# Autodesk Inventor assembly: ASY MSC 002 отстойник осветлитель
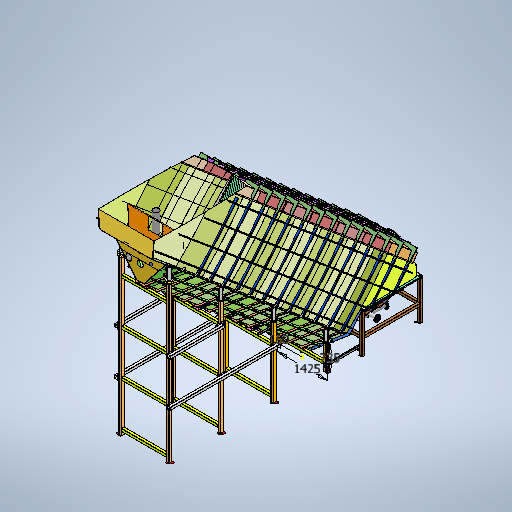
[picture p0: Inventor's stored thumbnail of the model, 512x512]
Saved by Autodesk Inventor 2025 (Build 290162010, 162A)
## iProperties
Created: 2024-09-05
Part Number: ASY MSC 002 отстойник осветлитель
Document SubType Name: Assembly
Designer: admin
Author: admin
## Documents named in this file (33)
- C:\Users\admin\YandexDisk-badmisterfox\домашниий пк\Inventor\Manturovo\Manturovo_Se-clar\ASY MSC 002 отстойник осветлитель.iam
- C:\Users\admin\YandexDisk-badmisterfox\домашниий пк\Inventor\Manturovo\Manturovo_Se-clar\ASY MSC 900.1 base frame.iam
- C:\Users\admin\YandexDisk-badmisterfox\домашниий пк\Inventor\Manturovo\Manturovo_Se-clar\ASY MSC 100 cone.iam
- C:\Users\admin\YandexDisk-badmisterfox\домашниий пк\Inventor\Manturovo\Manturovo_Se-clar\MSC 401 sheet lowerback.ipt
- C:\Users\admin\YandexDisk-badmisterfox\домашниий пк\Inventor\Manturovo\Manturovo_Se-clar\MSC 701 face 1.ipt
- C:\Users\admin\YandexDisk-badmisterfox\домашниий пк\Inventor\Manturovo\Manturovo_Se-clar\MSC 705 ridge 3.ipt
- C:\Users\admin\YandexDisk-badmisterfox\домашниий пк\Inventor\Manturovo\Manturovo_Se-clar\MSC 713 tube.ipt
- C:\Users\admin\YandexDisk-badmisterfox\домашниий пк\Inventor\Manturovo\Manturovo_Se-clar\ISO 5251 Bends 3D without straight ends(90 deg) DN150 11 11.ipt
- C:\Users\admin\YandexDisk-badmisterfox\домашниий пк\Inventor\Manturovo\Manturovo_Se-clar\MSC 408 stringer lowerback.ipt
- C:\Users\admin\YandexDisk-badmisterfox\домашниий пк\Inventor\Manturovo\Manturovo_Se-clar\MSC 703 face 2.ipt
- C:\Users\admin\YandexDisk-badmisterfox\домашниий пк\Inventor\Manturovo\Manturovo_Se-clar\MSC 702 face 3.ipt
- C:\Users\admin\YandexDisk-badmisterfox\домашниий пк\Inventor\Manturovo\Manturovo_Se-clar\MSC 704 face 4.ipt
- C:\Users\admin\YandexDisk-badmisterfox\домашниий пк\Inventor\Manturovo\Manturovo_Se-clar\ASY MSC 900.3 base frame.iam
- C:\Users\admin\YandexDisk-badmisterfox\домашниий пк\Inventor\Manturovo\Manturovo_Se-clar\Pillars\ASY MSC 900.5 base frame.iam
- C:\Users\admin\YandexDisk-badmisterfox\домашниий пк\Inventor\Manturovo\Manturovo_Se-clar\Pillars\ASY MSC 900.4  base frame.iam
- C:\Users\admin\YandexDisk-badmisterfox\домашниий пк\Inventor\Manturovo\Manturovo_Se-clar\Pillars\ASY MSC 900.6 base frame.iam
- C:\Users\admin\YandexDisk-badmisterfox\домашниий пк\Inventor\Manturovo\Manturovo_Se-clar\ASY MSC 200 BACK.iam
- C:\Users\admin\YandexDisk-badmisterfox\домашниий пк\Inventor\Manturovo\Manturovo_Se-clar\ASY MSC 300.2 LEFT BOARD.iam
- C:\Users\admin\YandexDisk-badmisterfox\домашниий пк\Inventor\Manturovo\Manturovo_Se-clar\ASY MSC 300.1 RIGHT BOARD.iam
- C:\Users\admin\YandexDisk-badmisterfox\домашниий пк\Inventor\Manturovo\Manturovo_Se-clar\ASY MSC 500 BELLY.iam
- C:\Users\admin\YandexDisk-badmisterfox\домашниий пк\Inventor\Manturovo\Manturovo_Se-clar\ASY MSC 900.2 support.iam
- C:\Users\admin\YandexDisk-badmisterfox\домашниий пк\Inventor\Manturovo\Manturovo_Se-clar\ASY MSC 600 cone exit back.iam
- C:\Users\admin\YandexDisk-badmisterfox\домашниий пк\Inventor\Manturovo\Manturovo_Se-clar\ASY MSC 800 gills.iam
- C:\Users\admin\YandexDisk-badmisterfox\домашниий пк\Inventor\Manturovo\Manturovo_Se-clar\ASY MSC 400 Accsess hatch.iam
- C:\Users\admin\YandexDisk-badmisterfox\домашниий пк\Inventor\Manturovo\Manturovo_Se-clar\MSC DIM 000 settler-clarifier.ipt
- C:\Users\admin\YandexDisk-badmisterfox\домашниий пк\Inventor\Manturovo\Manturovo_Se-clar\MSC DIM 001 frame.ipt
- C:\Users\admin\YandexDisk-badmisterfox\домашниий пк\Inventor\Manturovo\Manturovo_Se-clar\ASY MSC 900.7 base frame transverse.iam
- C:\Users\admin\YandexDisk-badmisterfox\домашниий пк\Inventor\Manturovo\Manturovo_Se-clar\ASY MSC 900.8 base frame transverse.iam
- C:\Users\admin\YandexDisk-badmisterfox\домашниий пк\Inventor\Manturovo\Manturovo_Se-clar\MSC 908 transverse pillar plate.ipt
- C:\Users\admin\YandexDisk-badmisterfox\домашниий пк\Inventor\Manturovo\Manturovo_Se-clar\Part2.ipt
- C:\Users\admin\YandexDisk-badmisterfox\домашниий пк\Inventor\Manturovo\Manturovo_Se-clar\MSC 900.9 base frame transverse.ipt
- C:\Users\admin\YandexDisk-badmisterfox\домашниий пк\Inventor\Manturovo\Manturovo_Se-clar\ASY MSC 700 water tray.iam
- C:\Users\admin\YandexDisk-badmisterfox\домашниий пк\Inventor\Manturovo\Manturovo_Se-clar\ASY 940 linkage.iam
## Components (51 placed, 32 different names)
1. MSC DIM 000 settler-clarifier:1
2. MSC DIM 001 frame:1
3. ASY MSC 900.1 base frame:1 [sub-assembly] — Flush:4, Mate:18, Flush:5, Mate:19, Mate:44, Mate:47, Mate:50, Flush:16
4. ASY MSC 100 cone:1 [sub-assembly] — Mate:19, Flush:6, Mate:29, Rigid:17
5. MSC 401 sheet lowerback:1 — Mate:29, Mate:30, Mate:31
6. MSC 701 face 1:1 — Rigid:4, Flush:9, Mate:35
7. MSC 705 ridge 3:1
8. MSC 713 tube:1 — Rigid:4
9. ISO 5251 Bends 3D without straight ends(90 deg) DN150 11:1
10. MSC 408 stringer lowerback:1
11. MSC 713 tube:2
12. MSC 703 face 2:1 — Flush:13, Flush:17, Mate:66
13. MSC 702 face 3:1 — Mate:34, Mate:35, Mate:36, Mate:66
14. MSC 704 face 4:1
15. MSC 408 stringer lowerback:2
16. ASY MSC 900.3 base frame:1 [sub-assembly] — Mate:23, Mate:24, Cylindrical:4, Mate:44, Mate:45, Rigid:26, Rigid:31, Rigid:32
17. ASY MSC 900.5 base frame:1 [sub-assembly] — Flush:11, Cylindrical:7, Cylindrical:8, Mate:46, Mate:48, Rigid:28
18. ASY MSC 900.4  base frame:1 [sub-assembly] — Mate:32, Mate:33, Mate:45, Mate:46, Rigid:27
19. ASY MSC 900.6 base frame:1 [sub-assembly] — Mate:38, Mate:39, Cylindrical:5, Cylindrical:6, Mate:47, Rigid:19, Rigid:20, Rigid:21, Rigid:22, Rigid:29
20. ASY MSC 200 BACK:1 [sub-assembly] — Flush:8, Mate:31
21. ASY MSC 300.2 LEFT BOARD:1 [sub-assembly] — Rigid:11, Mate:34
22. ASY MSC 300.1 RIGHT BOARD:1 [sub-assembly] — Rigid:10, Flush:17
23. ASY MSC 500 BELLY:1 [sub-assembly] — Flush:7, Mate:22, Mate:25, Rigid:10, Rigid:11, Mate:40, Mate:41, Mate:42, Mate:43
24. ASY MSC 900.2 support:1 [sub-assembly] — Cylindrical:8, Mate:40
25. ASY MSC 900.2 support:2 [sub-assembly]
26. ASY MSC 900.2 support:3 [sub-assembly] — Cylindrical:4, Mate:25
27. ASY MSC 900.2 support:4 [sub-assembly] — Cylindrical:6, Mate:42
28. ASY MSC 900.2 support:5 [sub-assembly]
29. ASY MSC 600 cone exit back:1 [sub-assembly] — Rigid:17
30. ASY MSC 800 gills:1 [sub-assembly] — Mate:22
31. ASY MSC 900.2 support:6 [sub-assembly] — Cylindrical:7, Mate:41
32. ASY MSC 900.2 support:7 [sub-assembly]
33. ASY MSC 400 Accsess hatch:1 [sub-assembly]
34. ASY MSC 900.2 support:8 [sub-assembly] — Cylindrical:5, Mate:43
35. ASY MSC 900.7 base frame transverse:1 [sub-assembly] — Rigid:19
36. ASY MSC 900.7 base frame transverse:2 [sub-assembly] — Rigid:20
37. ASY MSC 900.8 base frame transverse:1 [sub-assembly] — Rigid:21
38. ASY MSC 900.8 base frame transverse:2 [sub-assembly] — Rigid:22
39. MSC 908 transverse pillar plate:4 — Mate:50, Flush:16, Flush:18
40. Part2:1 — Rigid:26, Mate:51
41. MSC 900.9 base frame transverse:1 — Mate:51
42. Part2:2 — Rigid:27, Mate:59
43. MSC 900.9 base frame transverse:2 — Mate:59
44. Part2:3 — Rigid:28
45. MSC 900.9 base frame transverse:3
46. Part2:4 — Rigid:29
47. MSC 900.9 base frame transverse:4
48. ASY MSC 700 water tray:1 [sub-assembly]
49. ASY 940 linkage:1 [sub-assembly] — Rigid:32, Flush:18
50. MSC 908 transverse pillar plate:8
51. ASY 940 linkage:2 [sub-assembly] — Rigid:31
## Relationships (87: Mate 45, WeldJoint 19, Flush 14, CylindricalJoint 8, RevoluteJoint 1)
- [Mate]: ASY MSC 100 cone:1 ↔ MSC 401 sheet lowerback:1
- [WeldJoint]: MSC 713 tube:1 ↔ ISO 5251 Bends 3D without straight ends(90 deg) DN150 11:1
- [Mate]: ASY MSC 100 cone:1 ↔ MSC 408 stringer lowerback:1
- [RevoluteJoint]: ISO 5251 Bends 3D without straight ends(90 deg) DN150 11:1 ↔ MSC 713 tube:2
- Rigid:4 [WeldJoint]: MSC 701 face 1:1 ↔ MSC 713 tube:1
- [Mate]: ASY MSC 100 cone:1 ↔ MSC 408 stringer lowerback:2
- [Mate]: ASY MSC 500 BELLY:1 ↔ ASY MSC 600 cone exit back:1
- [Flush]: ASY MSC 900.1 base frame:1 ↔ ASY MSC 100 cone:1
- [WeldJoint]: MSC 705 ridge 3:1 ↔ ASY MSC 700 water tray:1
- [WeldJoint]: MSC 705 ridge 3:1 ↔ ASY MSC 700 water tray:1
- [Flush]: ASY MSC 500 BELLY:1 ↔ ASY MSC 600 cone exit back:1
- [Mate]: ASY MSC 500 BELLY:1 ↔ ASY MSC 800 gills:1
- [Mate]: MSC 701 face 1:1 ↔ ASY MSC 500 BELLY:1
- [Mate] (-5 mm): MSC 701 face 1:1 ↔ ASY MSC 500 BELLY:1
- [Mate] (3 mm): ASY MSC 500 BELLY:1 ↔ ASY MSC 900.2 support:2
- [Mate] (3 mm): ASY MSC 500 BELLY:1 ↔ ASY MSC 900.2 support:5
- [Mate] (3 mm): ASY MSC 500 BELLY:1 ↔ ASY MSC 900.2 support:7
- [CylindricalJoint]: ASY MSC 900.4  base frame:1 ↔ ASY MSC 900.2 support:5
- [CylindricalJoint]: ASY MSC 900.4  base frame:1 ↔ ASY MSC 900.2 support:2
- [Mate] (-2860 mm): ASY MSC 200 BACK:1 ↔ ASY MSC 500 BELLY:1
- [CylindricalJoint]: ASY MSC 900.3 base frame:1 ↔ ASY MSC 900.2 support:7
- [Flush]: ASY MSC 900.3 base frame:1 ↔ ASY MSC 900.4  base frame:1
- Flush:4: ASY MSC 900.1 base frame:1
- Mate:18 (4 mm): ASY MSC 900.1 base frame:1
- Flush:5: ASY MSC 900.1 base frame:1
- Mate:19: ASY MSC 900.1 base frame:1 ↔ ASY MSC 100 cone:1
- Flush:6: ASY MSC 100 cone:1
- Flush:7: ASY MSC 500 BELLY:1
- Flush:8: ASY MSC 200 BACK:1
- Mate:22: ASY MSC 500 BELLY:1 ↔ ASY MSC 800 gills:1
- Mate:23: ASY MSC 900.3 base frame:1
- Mate:24: ASY MSC 900.3 base frame:1
- Cylindrical:4: ASY MSC 900.3 base frame:1 ↔ ASY MSC 900.2 support:3
- Mate:25 (3 mm): ASY MSC 500 BELLY:1 ↔ ASY MSC 900.2 support:3
- Flush:9: MSC 701 face 1:1
- Mate:29: ASY MSC 100 cone:1 ↔ MSC 401 sheet lowerback:1
- Mate:30: MSC 401 sheet lowerback:1
- Mate:31: MSC 401 sheet lowerback:1 ↔ ASY MSC 200 BACK:1
- Rigid:10 [WeldJoint] (-25 mm): ASY MSC 300.1 RIGHT BOARD:1 ↔ ASY MSC 500 BELLY:1
- Rigid:11 [WeldJoint] (-25 mm): ASY MSC 300.2 LEFT BOARD:1 ↔ ASY MSC 500 BELLY:1
- Flush:11: ASY MSC 900.5 base frame:1
- Mate:32: ASY MSC 900.4  base frame:1
- Mate:33: ASY MSC 900.4  base frame:1
- Mate:34: MSC 702 face 3:1 ↔ ASY MSC 300.2 LEFT BOARD:1
- Mate:35: MSC 701 face 1:1 ↔ MSC 702 face 3:1
- [WeldJoint]: MSC 705 ridge 3:1 ↔ ASY MSC 700 water tray:1
- Mate:36: MSC 702 face 3:1
- Mate:38: ASY MSC 900.6 base frame:1
- Mate:39: ASY MSC 900.6 base frame:1
- Cylindrical:5: ASY MSC 900.6 base frame:1 ↔ ASY MSC 900.2 support:8
- Cylindrical:6: ASY MSC 900.6 base frame:1 ↔ ASY MSC 900.2 support:4
- Cylindrical:7: ASY MSC 900.5 base frame:1 ↔ ASY MSC 900.2 support:6
- Cylindrical:8: ASY MSC 900.5 base frame:1 ↔ ASY MSC 900.2 support:1
- Mate:40 (3 mm): ASY MSC 500 BELLY:1 ↔ ASY MSC 900.2 support:1
- Mate:41 (3 mm): ASY MSC 500 BELLY:1 ↔ ASY MSC 900.2 support:6
- Mate:42 (3 mm): ASY MSC 500 BELLY:1 ↔ ASY MSC 900.2 support:4
- Mate:43 (3 mm): ASY MSC 500 BELLY:1 ↔ ASY MSC 900.2 support:8
- Flush:13: MSC 703 face 2:1
- Mate:44 (820 mm): ASY MSC 900.1 base frame:1 ↔ ASY MSC 900.3 base frame:1
- Mate:45 (1430 mm): ASY MSC 900.3 base frame:1 ↔ ASY MSC 900.4  base frame:1
- Mate:46 (1430 mm): ASY MSC 900.5 base frame:1 ↔ ASY MSC 900.4  base frame:1
- Mate:47 (5315 mm): ASY MSC 900.1 base frame:1 ↔ ASY MSC 900.6 base frame:1
- Rigid:17 [WeldJoint]: ASY MSC 100 cone:1 ↔ ASY MSC 600 cone exit back:1
- Mate:48: ASY MSC 900.5 base frame:1
- Rigid:19 [WeldJoint]: ASY MSC 900.6 base frame:1 ↔ ASY MSC 900.7 base frame transverse:1
- Rigid:20 [WeldJoint]: ASY MSC 900.6 base frame:1 ↔ ASY MSC 900.7 base frame transverse:2
- Rigid:21 [WeldJoint]: ASY MSC 900.6 base frame:1 ↔ ASY MSC 900.8 base frame transverse:1
- Rigid:22 [WeldJoint]: ASY MSC 900.6 base frame:1 ↔ ASY MSC 900.8 base frame transverse:2
- Mate:50: ASY MSC 900.1 base frame:1 ↔ MSC 908 transverse pillar plate:4
- Rigid:26 [WeldJoint]: ASY MSC 900.3 base frame:1 ↔ Part2:1
- Mate:51: Part2:1 ↔ MSC 900.9 base frame transverse:1
- [Mate]: Part2:2 ↔ MSC 900.9 base frame transverse:2
- Rigid:27 [WeldJoint]: ASY MSC 900.4  base frame:1 ↔ Part2:2
- Mate:59: Part2:2 ↔ MSC 900.9 base frame transverse:2
- [Mate]: Part2:3 ↔ MSC 900.9 base frame transverse:3
- [Mate]: Part2:3 ↔ MSC 900.9 base frame transverse:3
- [Mate]: Part2:4 ↔ MSC 900.9 base frame transverse:4
- [Mate]: Part2:4 ↔ MSC 900.9 base frame transverse:4
- Rigid:28 [WeldJoint]: ASY MSC 900.5 base frame:1 ↔ Part2:3
- Rigid:29 [WeldJoint]: ASY MSC 900.6 base frame:1 ↔ Part2:4
- Flush:16 (-40 mm): ASY MSC 900.1 base frame:1 ↔ MSC 908 transverse pillar plate:4
- Flush:17: MSC 703 face 2:1 ↔ ASY MSC 300.1 RIGHT BOARD:1
- Mate:66: MSC 703 face 2:1 ↔ MSC 702 face 3:1
- [WeldJoint]: MSC 908 transverse pillar plate:8 ↔ ASY 940 linkage:2
- Rigid:31 [WeldJoint]: ASY MSC 900.3 base frame:1 ↔ ASY 940 linkage:2
- Rigid:32 [WeldJoint]: ASY MSC 900.3 base frame:1 ↔ ASY 940 linkage:1
- Flush:18: MSC 908 transverse pillar plate:4 ↔ ASY 940 linkage:1
## Named parameters: d131_d129 = 0 mm, d139_d131_d129 = 0 mm, d141_d138 = 0 mm, d142_d131_d129 = 0 mm, d144_d138 = 0 mm, d334_d122 = 0 mm
